# Autodesk Inventor assembly: Baterías
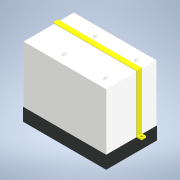
[picture p0: Inventor's stored thumbnail of the model, 180x180]
Saved by Autodesk Inventor 2022.1 (Build 261234000, 234)
## iProperties
Created: 2021-10-01
Part Number: Baterías
Document SubType Name: Assembly
Designer: seb_0
Author: seb_0
## Documents named in this file (4)
- C:\Users\seb_0\Desktop\PDM\ProyectoRobotPallet\Batería\Baterías.iam
- C:\Users\seb_0\Desktop\PDM\ProyectoRobotPallet\Batería\Batería.ipt
- C:\Users\seb_0\Desktop\PDM\ProyectoRobotPallet\Batería\Soporte_Batería.ipt
- C:\Users\seb_0\Desktop\PDM\ProyectoRobotPallet\Batería\Soporte_Batería2.ipt
## Components (4 placed, 3 different names)
1. Batería:1 — Coincidencia:1, Nivelación:1, Nivelación:2, Coincidencia:5, Coincidencia:6, Coincidencia:7
2. Batería:2 — Coincidencia:1, Nivelación:1, Nivelación:2, Coincidencia:2, Coincidencia:3, Coincidencia:4
3. Soporte_Batería:1 — Coincidencia:5, Coincidencia:6, Coincidencia:7, Coincidencia:8, Coincidencia:9, Coincidencia:10
4. Soporte_Batería2:1 — Coincidencia:8, Coincidencia:9, Coincidencia:10
## Relationships (12: Mate 10, Flush 2)
- Coincidencia:1 [Mate]: Batería:1 ↔ Batería:2
- Nivelación:1 [Flush]: Batería:1 ↔ Batería:2
- Nivelación:2 [Flush]: Batería:1 ↔ Batería:2
- Coincidencia:2 [Mate]: Batería:2
- Coincidencia:3 [Mate]: Batería:2
- Coincidencia:4 [Mate]: Batería:2
- Coincidencia:5 [Mate]: Batería:1 ↔ Soporte_Batería:1
- Coincidencia:6 [Mate]: Batería:1 ↔ Soporte_Batería:1
- Coincidencia:7 [Mate]: Batería:1 ↔ Soporte_Batería:1
- Coincidencia:8 [Mate]: Soporte_Batería:1 ↔ Soporte_Batería2:1
- Coincidencia:9 [Mate]: Soporte_Batería:1 ↔ Soporte_Batería2:1
- Coincidencia:10 [Mate]: Soporte_Batería:1 ↔ Soporte_Batería2:1
